# Autodesk Inventor assembly: Oktagon Zusammenbau
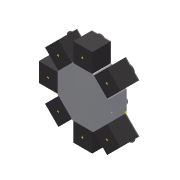
[picture p0: Inventor's stored thumbnail of the model, 180x180]
Saved by Autodesk Inventor 2018.2 (Build 222227000, 227)
## iProperties
Company: Fraunhofer ILT
Created: 2018-10-15
Part Number: Oktagon Zusammenbau
Material: geeigneten Werkstoff auswählen !
Document SubType Name: Assembly
Designer: N.Grubert
Title: =Description
Author: N.Grubert
## Documents named in this file (3)
- C:\Users\GRUBERT\Documents\COSIMA-Laserstar\CAD\Oktagon Zusammenbau.iam
- C:\Users\GRUBERT\Documents\COSIMA-Laserstar\CAD\Arduino_Oktagon.iam
- C:\Users\GRUBERT\Documents\COSIMA-Laserstar\CAD\Modul.iam
## Components (8 placed, 2 different names)
1. Arduino_Oktagon:1 [sub-assembly] — Passend:1, Passend:2, Passend:3, Passend:4, Passend:5, Passend:6, Passend:7, Passend:8, Passend:9, Passend:10, Fluchtend:9, Fluchtend:10, Fluchtend:11, Fluchtend:12, Fluchtend:13, Fluchtend:14, Fluchtend:15, Fluchtend:22
2. Modul:1 [sub-assembly] — Passend:4, Fluchtend:9, Fluchtend:17, Fluchtend:18
3. Modul:2 [sub-assembly] — Passend:5, Fluchtend:15, Fluchtend:18, Fluchtend:19
4. Modul:3 [sub-assembly] — Passend:6, Fluchtend:14, Fluchtend:19, Fluchtend:20
5. Modul:4 [sub-assembly] — Passend:7, Fluchtend:13, Fluchtend:20, Fluchtend:21
6. Modul:5 [sub-assembly] — Passend:8, Fluchtend:12, Fluchtend:21
7. Modul:6 [sub-assembly] — Passend:9, Fluchtend:11, Fluchtend:16, Fluchtend:22
8. Modul:7 [sub-assembly] — Passend:10, Fluchtend:10, Fluchtend:16, Fluchtend:17
## Relationships (24: Flush 14, Mate 10)
- Passend:1 [Mate]: Arduino_Oktagon:1
- Passend:2 [Mate]: Arduino_Oktagon:1
- Passend:3 [Mate]: Arduino_Oktagon:1
- Passend:4 [Mate]: Arduino_Oktagon:1 ↔ Modul:1
- Passend:5 [Mate]: Arduino_Oktagon:1 ↔ Modul:2
- Passend:6 [Mate]: Arduino_Oktagon:1 ↔ Modul:3
- Passend:7 [Mate]: Arduino_Oktagon:1 ↔ Modul:4
- Passend:8 [Mate]: Arduino_Oktagon:1 ↔ Modul:5
- Passend:9 [Mate]: Arduino_Oktagon:1 ↔ Modul:6
- Passend:10 [Mate]: Arduino_Oktagon:1 ↔ Modul:7
- Fluchtend:9 [Flush]: Arduino_Oktagon:1 ↔ Modul:1
- Fluchtend:10 [Flush]: Arduino_Oktagon:1 ↔ Modul:7
- Fluchtend:11 [Flush]: Arduino_Oktagon:1 ↔ Modul:6
- Fluchtend:12 [Flush]: Arduino_Oktagon:1 ↔ Modul:5
- Fluchtend:13 [Flush]: Arduino_Oktagon:1 ↔ Modul:4
- Fluchtend:14 [Flush]: Arduino_Oktagon:1 ↔ Modul:3
- Fluchtend:15 [Flush]: Arduino_Oktagon:1 ↔ Modul:2
- Fluchtend:16 [Flush]: Modul:6 ↔ Modul:7
- Fluchtend:17 [Flush]: Modul:1 ↔ Modul:7
- Fluchtend:18 [Flush]: Modul:1 ↔ Modul:2
- Fluchtend:19 [Flush]: Modul:2 ↔ Modul:3
- Fluchtend:20 [Flush]: Modul:3 ↔ Modul:4
- Fluchtend:21 [Flush]: Modul:4 ↔ Modul:5
- Fluchtend:22 [Flush]: Arduino_Oktagon:1 ↔ Modul:6
